# Autodesk Inventor assembly: Suction Cup 1764
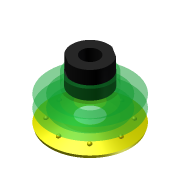
[picture p0: Inventor's stored thumbnail of the model, 180x180]
Saved by Autodesk Inventor 2011 (Build 150239000, 239)
## iProperties
Created: 2010-02-09
Part Number: Suction Cup 1764
Document SubType Name: Assembly
Designer: clee1
Author: clee1
## Documents named in this file (4)
- R:\2010-2011\CMO\Web Site\CADalog\Pneumatics\Suction Cup 1764\Suction Cup 1764.iam
- R:\2010-2011\CMO\Web Site\CADalog\Pneumatics\Suction Cup 1764\Suctin Cup Part 1 1764.ipt
- R:\2010-2011\CMO\Web Site\CADalog\Pneumatics\Suction Cup 1764\Suction Cup Part 2 1764.ipt
- R:\2010-2011\CMO\Web Site\CADalog\Pneumatics\Suction Cup 1764\Suction Cup Part 3 1764.ipt
## Components (3 placed, 3 different names)
1. Suctin Cup Part 1 1764:1 — Insert:1, Insert:2
2. Suction Cup Part 2 1764:1 — Insert:1
3. Suction Cup Part 3 1764:1 — Insert:2
## Relationships (2: Insert 2)
- Insert:1: Suctin Cup Part 1 1764:1 ↔ Suction Cup Part 2 1764:1
- Insert:2: Suctin Cup Part 1 1764:1 ↔ Suction Cup Part 3 1764:1
